# Autodesk Inventor assembly: Baugruppe1
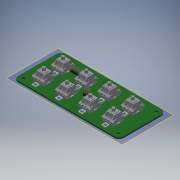
[picture p0: Inventor's stored thumbnail of the model, 180x180]
Saved by Autodesk Inventor 2019 (Build 230136000, 136)
## iProperties
Created: 2020-04-18
Part Number: Baugruppe1
Material: Generisch
Document SubType Name: Assembly
Designer: marc
Author: marc
## Documents named in this file (5)
- C:\Users\marc\Google Drive\Projekte\makroboard\makroboard_case\Baugruppe1.iam
- C:\Users\marc\Google Drive\Projekte\makroboard\makroboard_pcb\makroboard.iam
- C:\Users\marc\Google Drive\Projekte\makroboard\makroboard_case\case_bottom.ipt
- C:\Users\marc\Google Drive\Projekte\makroboard\makroboard_pcb\1054500101.ipt
- C:\Users\marc\Google Drive\Projekte\makroboard\makroboard_pcb\asm_mx_asm_PCB.iam
## Components (11 placed, 4 different names)
1. makroboard:1 [sub-assembly] — Fluchtend:1, Fluchtend:2, Starr:1, Starr:2, Starr:3, Starr:4, Starr:5, Starr:6, Starr:7, Drehbar:1, Starr:8
2. case_bottom:1 — Fluchtend:1, Fluchtend:2
3. 1054500101:1 — Starr:8
4. asm_mx_asm_PCB:1 [sub-assembly] — Starr:6
5. asm_mx_asm_PCB:2 [sub-assembly] — Starr:5
6. asm_mx_asm_PCB:3 [sub-assembly] — Starr:1
7. asm_mx_asm_PCB:4 [sub-assembly] — Starr:2
8. asm_mx_asm_PCB:5 [sub-assembly] — Starr:4
9. asm_mx_asm_PCB:6 [sub-assembly] — Drehbar:1
10. asm_mx_asm_PCB:7 [sub-assembly] — Starr:7
11. asm_mx_asm_PCB:8 [sub-assembly] — Starr:3
## Relationships (11: WeldJoint 8, Flush 2, RevoluteJoint 1)
- Fluchtend:1 [Flush]: makroboard:1 ↔ case_bottom:1
- Fluchtend:2 [Flush]: makroboard:1 ↔ case_bottom:1
- Starr:1 [WeldJoint] (-0.7 mm): makroboard:1 ↔ asm_mx_asm_PCB:3
- Starr:2 [WeldJoint]: makroboard:1 ↔ asm_mx_asm_PCB:4
- Starr:3 [WeldJoint]: makroboard:1 ↔ asm_mx_asm_PCB:8
- Starr:4 [WeldJoint]: makroboard:1 ↔ asm_mx_asm_PCB:5
- Starr:5 [WeldJoint]: makroboard:1 ↔ asm_mx_asm_PCB:2
- Starr:6 [WeldJoint]: makroboard:1 ↔ asm_mx_asm_PCB:1
- Starr:7 [WeldJoint]: makroboard:1 ↔ asm_mx_asm_PCB:7
- Drehbar:1 [RevoluteJoint] (-1.5 mm): makroboard:1 ↔ asm_mx_asm_PCB:6
- Starr:8 [WeldJoint]: makroboard:1 ↔ 1054500101:1
